# Autodesk Inventor assembly: Lift_Duct
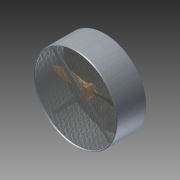
[picture p0: Inventor's stored thumbnail of the model, 180x180]
Saved by Autodesk Inventor 2011 SP1 (Build 150282100, 282)
## iProperties
Created: 2011-06-11
Part Number: Lift_Duct
Document SubType Name: Assembly
Designer: Andrew G. Meyer
Mass: 223.071 g
Surface Area: 3588.5 cm^2
Volume: 223.071 cm^3
Density: 1 g/cm^3
Author: Andrew G. Meyer
## Documents named in this file (7)
- C:\Users\Andrew G. Meyer\Documents\Inventor\Hovercraft\Lift_Duct.iam
- C:\Users\Andrew G. Meyer\Documents\Inventor\Hovercraft\Duct_Inner.ipt
- C:\Users\Andrew G. Meyer\Documents\Inventor\Hovercraft\Duct_Outer.ipt
- C:\Users\Andrew G. Meyer\Documents\Inventor\Hovercraft\Lift_Support.ipt
- C:\Users\Andrew G. Meyer\Documents\Inventor\Hovercraft\Duct_Guard.ipt
- C:\Users\Andrew G. Meyer\Documents\Inventor\Hovercraft\Lift_Motor.ipt
- C:\Users\Andrew G. Meyer\Documents\Inventor\Hovercraft\propellor.ipt
## Components (10 placed, 6 different names)
1. Duct_Inner:1 — Insert:1, Mate:4, Mate:5, Insert:2, Insert:3, Mate:8
2. Duct_Outer:1 — Insert:1
3. Lift_Support:1 — Flush:3, Mate:2, Flush:4, Mate:3, Mate:4, Mate:5, Mate:6
4. Lift_Support:2 — Mate:1, Flush:1, Flush:2, Mate:3
5. Lift_Support:3 — Flush:3, Mate:2, Flush:4, Flush:5
6. Lift_Support:4 — Mate:1, Flush:1, Flush:2, Flush:5, Mate:7, Mate:8
7. Duct_Guard:1 — Insert:2, Mate:6
8. Duct_Guard:2 — Insert:3
9. Lift_Motor:1 — Mate:7, Mate:9, Mate:10
10. propellor:1 — Mate:9, Mate:10
## Relationships (18: Mate 10, Flush 5, Insert 3)
- Insert:1: Duct_Inner:1 ↔ Duct_Outer:1
- Mate:1: Lift_Support:2 ↔ Lift_Support:4
- Flush:1: Lift_Support:2 ↔ Lift_Support:4
- Flush:2: Lift_Support:2 ↔ Lift_Support:4
- Flush:3: Lift_Support:1 ↔ Lift_Support:3
- Mate:2: Lift_Support:1 ↔ Lift_Support:3
- Flush:4: Lift_Support:1 ↔ Lift_Support:3
- Mate:3: Lift_Support:1 ↔ Lift_Support:2
- Flush:5: Lift_Support:3 ↔ Lift_Support:4
- Mate:4: Duct_Inner:1 ↔ Lift_Support:1
- Mate:5: Duct_Inner:1 ↔ Lift_Support:1
- Insert:2: Duct_Inner:1 ↔ Duct_Guard:1
- Mate:6 (12.7 mm): Lift_Support:1 ↔ Duct_Guard:1
- Insert:3: Duct_Inner:1 ↔ Duct_Guard:2
- Mate:7: Lift_Support:4 ↔ Lift_Motor:1
- Mate:8: Duct_Inner:1 ↔ Lift_Support:4
- Mate:9: Lift_Motor:1 ↔ propellor:1
- Mate:10: Lift_Motor:1 ↔ propellor:1
